# Autodesk Inventor assembly: battery_MIR
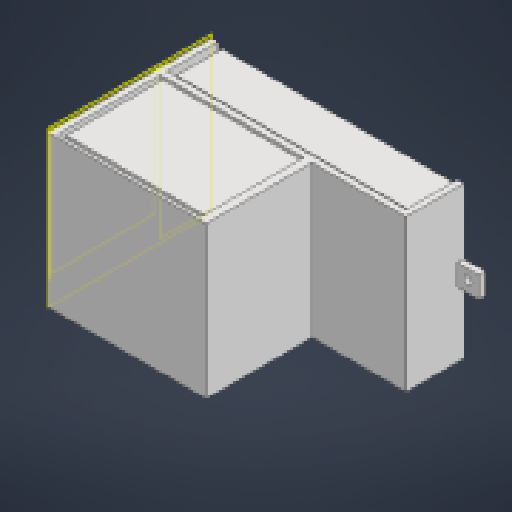
[picture p0: Inventor's stored thumbnail of the model, 512x512]
Saved by Autodesk Inventor 2026.1 (Build 301233020, 233B)
## iProperties
Created: 2025-11-26
Part Number: battery_MIR
Document SubType Name: Assembly
Designer: jaewook
Author: jaewook
## Documents named in this file (4)
- C:\Users\kjh19\Documents\Inventor\project\final\base_device\battery_MIR.iam
- C:\Users\kjh19\Documents\Inventor\project\final\base_device\battery_1_MIR.ipt
- C:\Users\kjh19\Documents\Inventor\project\final\base_device\battery_2_MIR.ipt
- C:\Users\kjh19\Documents\Inventor\project\final\battery_base_MIR.ipt
## Components (3 placed, 3 different names)
1. battery_1_MIR:1 — 강체:1
2. battery_2_MIR:1 — 강체:2
3. battery_base_MIR:1 — 강체:2, 강체:1
## Relationships (2: WeldJoint 2)
- 강체:2 [WeldJoint]: battery_2_MIR:1 ↔ battery_base_MIR:1
- 강체:1 [WeldJoint]: battery_1_MIR:1 ↔ battery_base_MIR:1
